# Autodesk Inventor assembly: Center Mount + odometry module
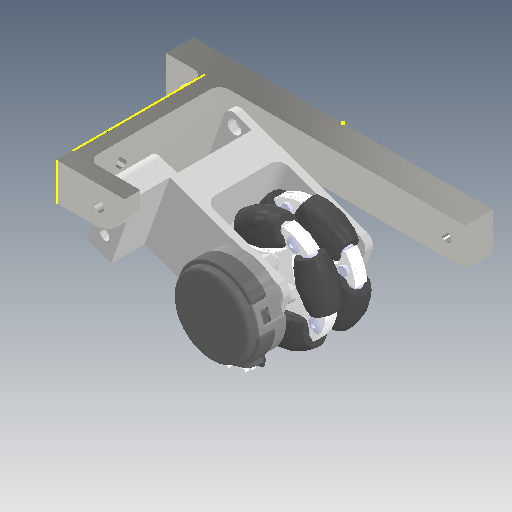
[picture p0: Inventor's stored thumbnail of the model, 512x512]
Saved by Autodesk Inventor 2020 (Build 240168000, 168)
## iProperties
Created: 2019-12-25
Part Number: Center Mount + odometry module
Document SubType Name: Assembly
Designer: ball
Author: ball
## Documents named in this file (4)
- C:\FTC\FTC8863CAD\2019 Robot\Odoemetry module\Center Mount + odometry module.iam
- C:\FTC\FTC8863CAD\2019 Robot\Odoemetry module\middleMountBracket.ipt
- C:\FTC\FTC8863CAD\2019 Robot\Odoemetry module\Odometry module.iam
- C:\FTC\FTC8863CAD\StepLibraries\Nuts\M4 NYLON-INSERT LOCKNUT.ipt
## Components (3 placed, 3 different names)
1. middleMountBracket:1 — Mate:1, Mate:2, Mate:3, Mate:4, Angle:1
2. Odometry module:1 [sub-assembly] — Mate:1, Mate:2
3. M4 NYLON-INSERT LOCKNUT:1 — Mate:3, Mate:4, Angle:1
## Relationships (5: Mate 4, Angle 1)
- Mate:1: middleMountBracket:1 ↔ Odometry module:1
- Mate:2 (1.27 mm): middleMountBracket:1 ↔ Odometry module:1
- Mate:3: middleMountBracket:1 ↔ M4 NYLON-INSERT LOCKNUT:1
- Mate:4: middleMountBracket:1 ↔ M4 NYLON-INSERT LOCKNUT:1
- Angle:1 (0 deg): middleMountBracket:1 ↔ M4 NYLON-INSERT LOCKNUT:1
